# Autodesk Inventor assembly: Lift - Top Motor Sprockets
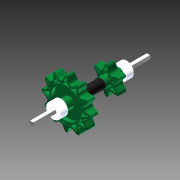
[picture p0: Inventor's stored thumbnail of the model, 180x180]
Saved by Autodesk Inventor 2012 (Build 160160000, 160)
## iProperties
Created: 2011-09-11
Part Number: Lift - Top Motor Sprockets
Document SubType Name: Assembly
Designer: Wade
Author: Wade
## Documents named in this file (7)
- C:\Users\Wade\Documents\1103 Robot - CAD Assembly\Lift - Top Motor Sprockets.iam
- C:\Users\Wade\Documents\24C VEX CAD Files\Drive Shafts\Drive Shaft (Square Bar) 4''.ipt
- C:\Users\Wade\Documents\24C VEX CAD Files\Gears & Pulleys\High Strength 12-Tooth Sprocket.ipt
- C:\Users\Wade\Documents\24C VEX CAD Files\Gears & Pulleys\High Strength 6-Tooth Sprocket.ipt
- C:\Users\Wade\Documents\24C VEX CAD Files\Washers & Spacers\Spacer (Nylon), 0.250''.ipt
- C:\Users\Wade\Documents\24C VEX CAD Files\Washers & Spacers\Spacer (Thick), 8mm.ipt
- C:\Users\Wade\Documents\24C VEX CAD Files\Washers & Spacers\Spacer (Thin), 4.6mm.ipt
## Components (8 placed, 6 different names)
1. Drive Shaft (Square Bar) 4'':1 — Mate:1, Mate:2, Mate:3, Mate:4, Flush:1, Flush:2
2. High Strength 12-Tooth Sprocket:1 — Mate:1, Mate:2, Mate:7, Mate:8, Mate:9, Mate:10
3. High Strength 6-Tooth Sprocket:1 — Mate:3, Mate:4, Mate:5, Mate:6, Mate:11, Mate:12
4. Spacer (Nylon), 0.250'':1 — Mate:5, Mate:6, Flush:2
5. Spacer (Nylon), 0.250'':2 — Mate:7, Mate:8, Flush:1
6. Spacer (Thick), 8mm:1 — Mate:9, Mate:10, Mate:14
7. Spacer (Thin), 4.6mm:1 — Mate:13, Mate:14
8. Spacer (Thick), 8mm:2 — Mate:11, Mate:12, Mate:13
## Relationships (16: Mate 14, Flush 2)
- Mate:1: Drive Shaft (Square Bar) 4'':1 ↔ High Strength 12-Tooth Sprocket:1
- Mate:2: Drive Shaft (Square Bar) 4'':1 ↔ High Strength 12-Tooth Sprocket:1
- Mate:3: Drive Shaft (Square Bar) 4'':1 ↔ High Strength 6-Tooth Sprocket:1
- Mate:4: Drive Shaft (Square Bar) 4'':1 ↔ High Strength 6-Tooth Sprocket:1
- Mate:5: High Strength 6-Tooth Sprocket:1 ↔ Spacer (Nylon), 0.250'':1
- Mate:6: High Strength 6-Tooth Sprocket:1 ↔ Spacer (Nylon), 0.250'':1
- Mate:7: High Strength 12-Tooth Sprocket:1 ↔ Spacer (Nylon), 0.250'':2
- Mate:8: High Strength 12-Tooth Sprocket:1 ↔ Spacer (Nylon), 0.250'':2
- Mate:9: High Strength 12-Tooth Sprocket:1 ↔ Spacer (Thick), 8mm:1
- Mate:10: High Strength 12-Tooth Sprocket:1 ↔ Spacer (Thick), 8mm:1
- Mate:11: High Strength 6-Tooth Sprocket:1 ↔ Spacer (Thick), 8mm:2
- Mate:12: High Strength 6-Tooth Sprocket:1 ↔ Spacer (Thick), 8mm:2
- Mate:13: Spacer (Thin), 4.6mm:1 ↔ Spacer (Thick), 8mm:2
- Mate:14 (-1.27 mm): Spacer (Thick), 8mm:1 ↔ Spacer (Thin), 4.6mm:1
- Flush:1 (-19.05 mm): Drive Shaft (Square Bar) 4'':1 ↔ Spacer (Nylon), 0.250'':2
- Flush:2 (19.05 mm): Drive Shaft (Square Bar) 4'':1 ↔ Spacer (Nylon), 0.250'':1
